# Autodesk Inventor assembly: slik_clamp_head38
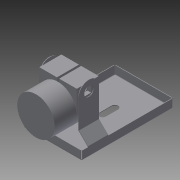
[picture p0: Inventor's stored thumbnail of the model, 180x180]
Saved by Autodesk Inventor 2013 (Build 170138000, 138)
## iProperties
Created: 2013-01-30
Part Number: slik_clamp_head38
Document SubType Name: Assembly
Designer: Mahisorn
Author: Mahisorn
## Documents named in this file (4)
- E:\mahisorn\documents\hg-ros-pkg\cad\gripper\slik_clamp_head38.iam
- E:\mahisorn\documents\hg-ros-pkg\cad\gripper\slik_clamp_head38_stud.ipt
- E:\mahisorn\documents\hg-ros-pkg\cad\gripper\slik_clamp_head38_collar.ipt
- E:\mahisorn\documents\hg-ros-pkg\cad\gripper\slik_clamp_head38_plate.ipt
## Components (3 placed, 3 different names)
1. slik_clamp_head38_stud:1 — Insert:1
2. slik_clamp_head38_collar:1 — Insert:1, Insert:2
3. slik_clamp_head38_plate:1 — Insert:2
## Relationships (2: Insert 2)
- Insert:1: slik_clamp_head38_stud:1 ↔ slik_clamp_head38_collar:1
- Insert:2 (0.5 mm): slik_clamp_head38_collar:1 ↔ slik_clamp_head38_plate:1
